# Autodesk Inventor assembly: NixieClock
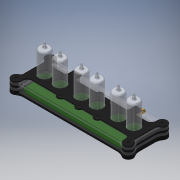
[picture p0: Inventor's stored thumbnail of the model, 180x180]
Saved by Autodesk Inventor 2017 (Build 210142000, 142)
## iProperties
Created: 2017-04-18
Part Number: NixieClock
Document SubType Name: Assembly
Designer: jeffkub
Author: jeffkub
## Documents named in this file (9)
- C:\Projects\nixie-clock\mechanical\NixieClock.iam
- C:\Projects\nixie-clock\mechanical\Base1.ipt
- C:\Projects\nixie-clock\mechanical\Base2.ipt
- C:\Projects\nixie-clock\mechanical\PCB.iam
- C:\Projects\nixie-clock\mechanical\Side.iam
- C:\Projects\nixie-clock\mechanical\Top.ipt
- C:\Projects\nixie-clock\mechanical\Cover.ipt
- C:\Projects\nixie-clock\mechanical\Front.ipt
- C:\Projects\nixie-clock\mechanical\Back.ipt
## Components (9 placed, 8 different names)
1. Base1:1 — Flush:1, Flush:2, Flush:3, Mate:1
2. Base2:1 — Mate:1, Flush:4, Flush:5, Mate:2, Mate:4, Mate:6, Mate:8, Mate:9, Mate:11, Mate:14
3. PCB:1 [sub-assembly] — Mate:2, Flush:6, Flush:7
4. Side:1 [sub-assembly] — Mate:4, Angle:1, Mate:7, Flush:11, Mate:8, Mate:13
5. Side:2 [sub-assembly] — Mate:6, Angle:2, Mate:9, Mate:15
6. Top:1 — Flush:8, Flush:9, Mate:7, Mate:10
7. Cover:1 — Flush:10, Flush:12, Flush:13, Mate:10
8. Front:1 — Mate:11, Mate:13, Flush:14
9. Back:1 — Flush:15, Mate:14, Mate:15
## Relationships (29: Flush 15, Mate 12, Angle 2)
- Flush:1: Base1:1
- Flush:2: Base1:1
- Flush:3: Base1:1
- Mate:1: Base1:1 ↔ Base2:1
- Flush:4: Base2:1
- Flush:5: Base2:1
- Mate:2: Base2:1 ↔ PCB:1
- Flush:6: PCB:1
- Flush:7: PCB:1
- Mate:4: Base2:1 ↔ Side:1
- Angle:1 (0 deg): Side:1
- Mate:6: Base2:1 ↔ Side:2
- Angle:2 (180 deg): Side:2
- Flush:8: Top:1
- Flush:9: Top:1
- Mate:7: Side:1 ↔ Top:1
- Flush:10: Cover:1
- Flush:11: Side:1
- Mate:8: Base2:1 ↔ Side:1
- Mate:9: Base2:1 ↔ Side:2
- Flush:12: Cover:1
- Flush:13: Cover:1
- Mate:10: Top:1 ↔ Cover:1
- Mate:11 (0.05 mm): Base2:1 ↔ Front:1
- Mate:13 (0.1 mm): Side:1 ↔ Front:1
- Flush:14: Front:1
- Flush:15: Back:1
- Mate:14 (0.05 mm): Base2:1 ↔ Back:1
- Mate:15 (0.1 mm): Side:2 ↔ Back:1
